# Autodesk Inventor assembly: Full_Design
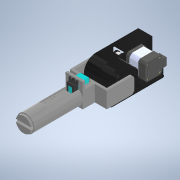
[picture p0: Inventor's stored thumbnail of the model, 180x180]
Saved by Autodesk Inventor 2022 (Build 260153000, 153)
## iProperties
Created: 2022-03-12
Part Number: Full_Design
Document SubType Name: Assembly
Designer: Mlees
Author: Mlees
## Documents named in this file (23)
- C:\Users\Mlees\Desktop\504Engineering\Stepper-Servo_Based_Robotic_Arm\Designs\Version_8\Full_Design.iam
- C:\Users\Mlees\Desktop\504Engineering\Stepper-Servo_Based_Robotic_Arm\Designs\Version_7\Created_Parts\Combined_Gear_Box_Modified_3.ipt
- C:\Users\Mlees\Desktop\504Engineering\Stepper-Servo_Based_Robotic_Arm\Designs\Version_7\Created_Parts\Gear_Cover_modified.ipt
- C:\Users\Mlees\Desktop\504Engineering\Stepper-Servo_Based_Robotic_Arm\Designs\Version_7\Created_Parts\Planet_Carrier_Modifed_with_sun_gear.ipt
- C:\Users\Mlees\Desktop\504Engineering\Stepper-Servo_Based_Robotic_Arm\Designs\Version_7\Created_Parts\Plamet_Carrier.ipt
- C:\Users\Mlees\Desktop\504Engineering\Stepper-Servo_Based_Robotic_Arm\Designs\Version_7\Created_Parts\Belt_Bearing_Holder.ipt
- C:\Users\Mlees\Desktop\504Engineering\Stepper-Servo_Based_Robotic_Arm\Designs\Version_7\Created_Parts\Belt_Bearing_Holder_p2.ipt
- C:\Users\Mlees\Desktop\504Engineering\Stepper-Servo_Based_Robotic_Arm\Designs\Version_7\Created_Parts\Belt_Tension_Bearing.ipt
- C:\Users\Mlees\Desktop\504Engineering\Stepper-Servo_Based_Robotic_Arm\Designs\Version_7\Created_Parts\24_Teeth_Sun_Gear.ipt
- C:\Users\Mlees\Desktop\504Engineering\Stepper-Servo_Based_Robotic_Arm\Designs\Version_7\Created_Parts\36_Teeth_Planet_Gear.ipt
- C:\Users\Mlees\Desktop\504Engineering\Stepper-Servo_Based_Robotic_Arm\Designs\Version_7\Created_Parts\Metal_AttachmentBracket.ipt
- C:\Users\Mlees\Desktop\504Engineering\Stepper-Servo_Based_Robotic_Arm\Designs\Version_7\Created_Parts\Twist_Rod.ipt
- C:\Users\Mlees\Desktop\504Engineering\Stepper-Servo_Based_Robotic_Arm\Designs\Version_7\Downloaded_Parts\9403T15_Tight-Tolerance High-Strength 7075 Aluminum Rod.ipt
- C:\Users\Mlees\Desktop\504Engineering\Stepper-Servo_Based_Robotic_Arm\Designs\Version_7\Downloaded_Parts\GT2 20T Drive Pulley.ipt
- C:\Users\Mlees\Desktop\504Engineering\Stepper-Servo_Based_Robotic_Arm\Designs\Version_7\Downloaded_Parts\GT2 60T Drive Pulley.ipt
- C:\Users\Mlees\Desktop\504Engineering\Stepper-Servo_Based_Robotic_Arm\Designs\Version_7\Downloaded_Parts\124125202-9-stp-mtr-17040w\stp-mtr-17040w.ipt
- C:\Users\Mlees\Desktop\504Engineering\Stepper-Servo_Based_Robotic_Arm\Designs\Version_7\Created_Parts\Combined_Gear_Box_Modified_2.ipt
- C:\Users\Mlees\Desktop\504Engineering\Stepper-Servo_Based_Robotic_Arm\Designs\Version_7\Created_Parts\Tilt_Bracket_Output_2.ipt
- C:\Users\Mlees\Desktop\504Engineering\Stepper-Servo_Based_Robotic_Arm\Designs\Version_7\Created_Parts\Tilt_Bracket_Output_2_Lid.ipt
- C:\Users\Mlees\Desktop\504Engineering\Stepper-Servo_Based_Robotic_Arm\Designs\Version_7\Created_Parts\Twist_Attachment_To_Servo_Horn.ipt
- C:\Users\Mlees\Desktop\504Engineering\Stepper-Servo_Based_Robotic_Arm\Designs\Version_7\Created_Parts\Twist_Servo_Horn.ipt
- C:\Users\Mlees\Desktop\504Engineering\Stepper-Servo_Based_Robotic_Arm\Designs\Version_7\Downloaded_Parts\uploads_files_140274_ServoSW-1211SG.ipt
- C:\Users\Mlees\Desktop\504Engineering\Stepper-Servo_Based_Robotic_Arm\Designs\Version_8\Created_Parts\Claw_Attachment.ipt
## Components (28 placed, 22 different names)
1. Combined_Gear_Box_Modified_3:1 — Rigid:1, Rigid:4, Rotational:12, Rotational:16
2. Gear_Cover_modified:1 — Rotational:15
3. Planet_Carrier_Modifed_with_sun_gear:1 — Rotational:4, Rotational:5, Rotational:6, Rotation:2, Rotational:13, Rotational:14
4. Plamet_Carrier:1 — Rotational:7, Rotational:8, Rotational:9, Rotational:14
5. Belt_Bearing_Holder:1 — Rotational:10, Rigid:6, Rotational:12
6. Belt_Bearing_Holder_p2:1 — Rigid:6
7. Belt_Tension_Bearing:1 — Rotational:11
8. Belt_Tension_Bearing:2 — Rotational:10, Rotational:11
9. 24_Teeth_Sun_Gear:1 — Rigid:2, Rotation:2, Rotational:13
10. 36_Teeth_Planet_Gear:1 — Rotational:4
11. 36_Teeth_Planet_Gear:2 — Rotational:5
12. 36_Teeth_Planet_Gear:3 — Rotational:6
13. Metal_AttachmentBracket:1 — Rigid:5, Rigid:1
14. 9403T15_Tight-Tolerance High-Strength 7075 Aluminum Rod:1 — Rigid:2, Rigid:3, Rotation:1
15. GT2 20T Drive Pulley:1 — Rotational:2, Rotation:1
16. GT2 60T Drive Pulley:1 — Rigid:3, Rotational:3
17. stp-mtr-17040w:1 — Rigid:5, Rotational:2
18. 36_Teeth_Planet_Gear:4 — Rotational:7
19. 36_Teeth_Planet_Gear:5 — Rotational:8
20. 36_Teeth_Planet_Gear:6 — Rotational:9
21. Combined_Gear_Box_Modified_2:1 — Rigid:4, Rotational:3, Rotational:15
22. Tilt_Bracket_Output_2:1 — Rotational:16, Rotational:17, Rigid:9
23. Tilt_Bracket_Output_2_Lid:1 — Rigid:10
24. Twist_Attachment_To_Servo_Horn:1 — Rigid:8, Rotational:17
25. Twist_Rod:1 — Rigid:7, Rigid:8
26. Twist_Servo_Horn:1 — Rotational:18
27. uploads_files_140274_ServoSW-1211SG:1 — Rigid:9, Rotational:18, Rigid:10
28. Claw_Attachment:1 — Rigid:7
## Relationships (29: RevoluteJoint 17, WeldJoint 10, RelateRotation 2)
- Rigid:5 [WeldJoint]: Metal_AttachmentBracket:1 ↔ stp-mtr-17040w:1
- Rigid:1 [WeldJoint]: Combined_Gear_Box_Modified_3:1 ↔ Metal_AttachmentBracket:1
- Rigid:2 [WeldJoint]: 24_Teeth_Sun_Gear:1 ↔ 9403T15_Tight-Tolerance High-Strength 7075 Aluminum Rod:1
- Rigid:3 [WeldJoint]: 9403T15_Tight-Tolerance High-Strength 7075 Aluminum Rod:1 ↔ GT2 60T Drive Pulley:1
- Rigid:4 [WeldJoint]: Combined_Gear_Box_Modified_3:1 ↔ Combined_Gear_Box_Modified_2:1
- Rotational:2 [RevoluteJoint]: GT2 20T Drive Pulley:1 ↔ stp-mtr-17040w:1
- Rotational:3 [RevoluteJoint]: GT2 60T Drive Pulley:1 ↔ Combined_Gear_Box_Modified_2:1
- Rotation:1 [RelateRotation] (1 ul): 9403T15_Tight-Tolerance High-Strength 7075 Aluminum Rod:1 ↔ GT2 20T Drive Pulley:1
- Rotational:4 [RevoluteJoint]: Planet_Carrier_Modifed_with_sun_gear:1 ↔ 36_Teeth_Planet_Gear:1
- Rotational:5 [RevoluteJoint]: Planet_Carrier_Modifed_with_sun_gear:1 ↔ 36_Teeth_Planet_Gear:2
- Rotational:6 [RevoluteJoint]: Planet_Carrier_Modifed_with_sun_gear:1 ↔ 36_Teeth_Planet_Gear:3
- Rotational:7 [RevoluteJoint]: Plamet_Carrier:1 ↔ 36_Teeth_Planet_Gear:4
- Rotational:8 [RevoluteJoint]: Plamet_Carrier:1 ↔ 36_Teeth_Planet_Gear:5
- Rotational:9 [RevoluteJoint]: Plamet_Carrier:1 ↔ 36_Teeth_Planet_Gear:6
- Rotational:10 [RevoluteJoint]: Belt_Bearing_Holder:1 ↔ Belt_Tension_Bearing:2
- Rotational:11 [RevoluteJoint]: Belt_Tension_Bearing:1 ↔ Belt_Tension_Bearing:2
- Rigid:6 [WeldJoint]: Belt_Bearing_Holder:1 ↔ Belt_Bearing_Holder_p2:1
- Rotational:12 [RevoluteJoint] (10 mm): Combined_Gear_Box_Modified_3:1 ↔ Belt_Bearing_Holder:1
- Rotation:2 [RelateRotation] (1 ul): Planet_Carrier_Modifed_with_sun_gear:1 ↔ 24_Teeth_Sun_Gear:1
- Rotational:13 [RevoluteJoint]: Planet_Carrier_Modifed_with_sun_gear:1 ↔ 24_Teeth_Sun_Gear:1
- Rotational:14 [RevoluteJoint]: Planet_Carrier_Modifed_with_sun_gear:1 ↔ Plamet_Carrier:1
- Rotational:15 [RevoluteJoint]: Gear_Cover_modified:1 ↔ Combined_Gear_Box_Modified_2:1
- Rotational:16 [RevoluteJoint]: Combined_Gear_Box_Modified_3:1 ↔ Tilt_Bracket_Output_2:1
- Rigid:7 [WeldJoint]: Twist_Rod:1 ↔ Claw_Attachment:1
- Rigid:8 [WeldJoint]: Twist_Attachment_To_Servo_Horn:1 ↔ Twist_Rod:1
- Rotational:17 [RevoluteJoint]: Tilt_Bracket_Output_2:1 ↔ Twist_Attachment_To_Servo_Horn:1
- Rigid:9 [WeldJoint]: Tilt_Bracket_Output_2:1 ↔ uploads_files_140274_ServoSW-1211SG:1
- Rotational:18 [RevoluteJoint]: Twist_Servo_Horn:1 ↔ uploads_files_140274_ServoSW-1211SG:1
- Rigid:10 [WeldJoint]: Tilt_Bracket_Output_2_Lid:1 ↔ uploads_files_140274_ServoSW-1211SG:1
